# Autodesk Inventor assembly: ESTACION_TOTAL
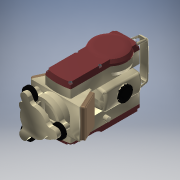
[picture p0: Inventor's stored thumbnail of the model, 180x180]
Saved by Autodesk Inventor 2016 (Build 200138000, 138)
## iProperties
Created: 2016-03-24
Part Number: ESTACION_TOTAL
Material: Genérico
Document SubType Name: Assembly
Designer: Usuario1
Author: Usuario1
## Documents named in this file (21)
- C:\Users\Usuario1\Desktop\REPOSITORIO3D\ESTACION TOTAL\ESTACION_TOTAL.iam
- C:\Users\Usuario1\Desktop\REPOSITORIO3D\ESTACION TOTAL\ET1.ipt
- C:\Users\Usuario1\Desktop\REPOSITORIO3D\ESTACION TOTAL\ET2.ipt
- C:\Users\Usuario1\Desktop\REPOSITORIO3D\ESTACION TOTAL\ET3.ipt
- C:\Users\Usuario1\Desktop\REPOSITORIO3D\ESTACION TOTAL\ET4.ipt
- C:\Users\Usuario1\Desktop\REPOSITORIO3D\ESTACION TOTAL\ET5.ipt
- C:\Users\Usuario1\Desktop\REPOSITORIO3D\ESTACION TOTAL\ET9.ipt
- C:\Users\Usuario1\Desktop\REPOSITORIO3D\ESTACION TOTAL\ET8.ipt
- C:\Users\Usuario1\Desktop\REPOSITORIO3D\ESTACION TOTAL\ET11.ipt
- C:\Users\Usuario1\Desktop\REPOSITORIO3D\ESTACION TOTAL\ET10.ipt
- C:\Users\Usuario1\Desktop\REPOSITORIO3D\ESTACION TOTAL\ET7.ipt
- C:\Users\Usuario1\Desktop\REPOSITORIO3D\ESTACION TOTAL\ET6.ipt
- C:\Users\Usuario1\Desktop\REPOSITORIO3D\ESTACION TOTAL\ET13.ipt
- C:\Users\Usuario1\Desktop\REPOSITORIO3D\ESTACION TOTAL\ET12.ipt
- C:\Users\Usuario1\Desktop\REPOSITORIO3D\ESTACION TOTAL\ET14.ipt
- C:\Users\Usuario1\Desktop\REPOSITORIO3D\ESTACION TOTAL\ET15.ipt
- C:\Users\Usuario1\Desktop\REPOSITORIO3D\ESTACION TOTAL\ET16.ipt
- C:\Users\Usuario1\Desktop\REPOSITORIO3D\ESTACION TOTAL\ET17.ipt
- C:\Users\Usuario1\Desktop\REPOSITORIO3D\ESTACION TOTAL\ET18.ipt
- C:\Users\Usuario1\Desktop\REPOSITORIO3D\ESTACION TOTAL\ET19.ipt
- C:\Users\Usuario1\Desktop\REPOSITORIO3D\ESTACION TOTAL\ET20.ipt
## Components (22 placed, 20 different names)
1. ET1:1 — De rotación:1, De rotación:2, De rotación:3
2. ET2:1 — De rotación:1
3. ET2:2 — De rotación:2, De rotación:4
4. ET2:3 — De rotación:3
5. ET3:1 — De rotación:4, De rotación:5
6. ET4:1 — De rotación:5, De rotación:6
7. ET5:1 — De rotación:6, Coincidencia:4, Coincidencia:5, Coincidencia:9, Coincidencia:11, Coincidencia:12, Coincidencia:13, Coincidencia:14
8. ET9:1 — Coincidencia:4, Coincidencia:5, Coincidencia:7, Coincidencia:8, Coincidencia:15
9. ET8:1 — Coincidencia:7, Coincidencia:8
10. ET11:1 — Coincidencia:9, Coincidencia:10
11. ET10:1 — Coincidencia:10
12. ET7:1 — Coincidencia:11
13. ET6:1 — Coincidencia:12
14. ET13:1 — Coincidencia:13, Coincidencia:14
15. ET12:1 — Coincidencia:15
16. ET14:1
17. ET15:1
18. ET16:1
19. ET17:1
20. ET18:1
21. ET19:1
22. ET20:1
## Relationships (17: Mate 11, RevoluteJoint 6)
- De rotación:1 [RevoluteJoint]: ET1:1 ↔ ET2:1
- De rotación:2 [RevoluteJoint]: ET1:1 ↔ ET2:2
- De rotación:3 [RevoluteJoint]: ET1:1 ↔ ET2:3
- De rotación:4 [RevoluteJoint]: ET2:2 ↔ ET3:1
- De rotación:5 [RevoluteJoint]: ET3:1 ↔ ET4:1
- De rotación:6 [RevoluteJoint]: ET4:1 ↔ ET5:1
- Coincidencia:4 [Mate]: ET5:1 ↔ ET9:1
- Coincidencia:5 [Mate]: ET5:1 ↔ ET9:1
- Coincidencia:7 [Mate]: ET9:1 ↔ ET8:1
- Coincidencia:8 [Mate]: ET9:1 ↔ ET8:1
- Coincidencia:9 [Mate]: ET5:1 ↔ ET11:1
- Coincidencia:10 [Mate]: ET11:1 ↔ ET10:1
- Coincidencia:11 [Mate]: ET5:1 ↔ ET7:1
- Coincidencia:12 [Mate]: ET5:1 ↔ ET6:1
- Coincidencia:13 [Mate]: ET5:1 ↔ ET13:1
- Coincidencia:14 [Mate]: ET5:1 ↔ ET13:1
- Coincidencia:15 [Mate]: ET9:1 ↔ ET12:1
